# Autodesk Inventor assembly: USB Cable B Male to B Female 90 degrees_Assembly
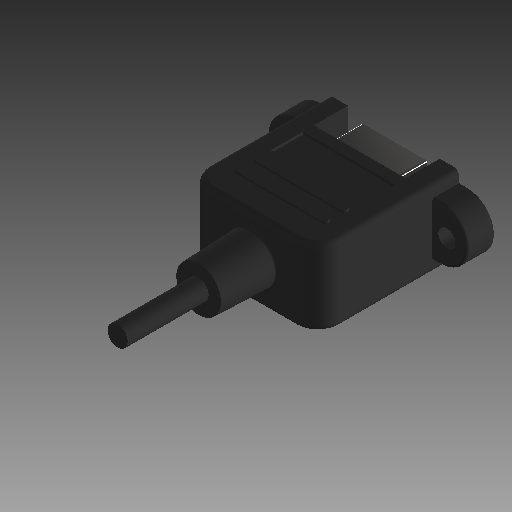
[picture p0: Inventor's stored thumbnail of the model, 512x512]
Saved by Autodesk Inventor 2019 (Build 230136000, 136)
## iProperties
Created: 2017-10-16
Part Number: USB Cable B Male to B Female 90 degrees_Assembly
Document SubType Name: Assembly
Designer: admin
Author: admin
## Documents named in this file (3)
- I:\CMR4GR\Documents\Inventor\ESTOP V2\USB Cable B Male to B Female 90 degrees_Assembly.iam
- I:\CMR4GR\Documents\Inventor\ESTOP V2\USB Cable B Male to B Female 90 degrees.ipt
- I:\CMR4GR\Documents\Inventor\ESTOP V2\USB B Female Port.ipt
## Components (2 placed, 2 different names)
1. USB Cable B Male to B Female 90 degrees:1 — Flush:1, Flush:2, Mate:1
2. USB B Female Port:1 — Flush:1, Flush:2, Mate:1
## Relationships (3: Flush 2, Mate 1)
- Flush:1 (1.6135 mm): USB Cable B Male to B Female 90 degrees:1 ↔ USB B Female Port:1
- Flush:2 (-6.41 mm): USB Cable B Male to B Female 90 degrees:1 ↔ USB B Female Port:1
- Mate:1 (2.4675 mm): USB Cable B Male to B Female 90 degrees:1 ↔ USB B Female Port:1
